# Autodesk Inventor assembly: Link_01_Assembly_V02
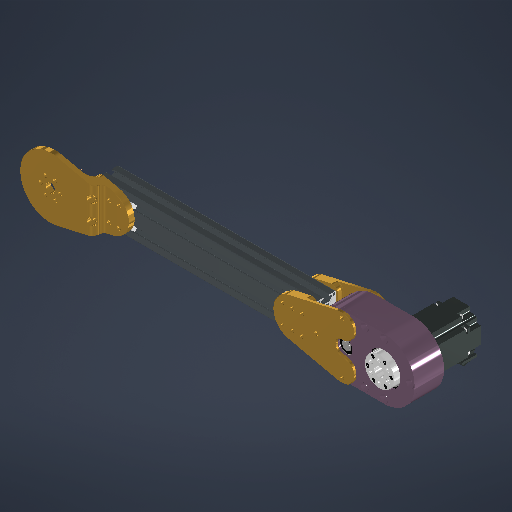
[picture p0: Inventor's stored thumbnail of the model, 512x512]
Saved by Autodesk Inventor 2026 (Build 300175000, 175)
## iProperties
Created: 2025-12-01
Part Number: Link_01_Assembly_V02
Document SubType Name: Assembly
Designer: DanielFGarzon
Mass: 2273.35 g
Surface Area: 4707.46 cm^2
Volume: 1022.63 cm^3
Density: 2.22304 g/cm^3
Author: DanielFGarzon
## Documents named in this file (5)
- D:\POLIMI\3RD SEMESTER\Industrial Robotics\Project\Mine\Link_01_Assembly_V02.iam
- D:\POLIMI\3RD SEMESTER\Industrial Robotics\Project\Mine\RotationalConector_30x60.ipt
- D:\POLIMI\3RD SEMESTER\Industrial Robotics\Project\Mine\Link_01_V02.ipt
- D:\POLIMI\3RD SEMESTER\Industrial Robotics\Project\Mine\RigidConector_30x60.ipt
- D:\POLIMI\3RD SEMESTER\Industrial Robotics\Project\Mine\Reducer.iam
## Components (5 placed, 4 different names)
1. RotationalConector_30x60:1 — Mate:1, Mate:2, Mate:3, Mate:4
2. Link_01_V02:1 — Mate:2, Mate:3, Mate:4, Mate:5, Mate:6, Mate:7, Mate:8, Mate:9, Mate:10, Flush:2, Mate:15
3. RigidConector_30x60:1 — Mate:5, Mate:6, Mate:7, Mate:11, Mate:13
4. RigidConector_30x60:2 — Mate:8, Mate:9, Mate:10, Mate:12
5. Reducer:1 [sub-assembly] — Mate:11, Mate:12, Mate:13
## Relationships (16: Mate 15, Flush 1)
- Mate:1: RotationalConector_30x60:1
- Mate:2: RotationalConector_30x60:1 ↔ Link_01_V02:1
- Mate:3: RotationalConector_30x60:1 ↔ Link_01_V02:1
- Mate:4: RotationalConector_30x60:1 ↔ Link_01_V02:1
- Mate:5: Link_01_V02:1 ↔ RigidConector_30x60:1
- Mate:6: Link_01_V02:1 ↔ RigidConector_30x60:1
- Mate:7: Link_01_V02:1 ↔ RigidConector_30x60:1
- Mate:8: Link_01_V02:1 ↔ RigidConector_30x60:2
- Mate:9: Link_01_V02:1 ↔ RigidConector_30x60:2
- Mate:10: Link_01_V02:1 ↔ RigidConector_30x60:2
- Mate:11: RigidConector_30x60:1 ↔ Reducer:1
- Mate:12: RigidConector_30x60:2 ↔ Reducer:1
- Mate:13: RigidConector_30x60:1 ↔ Reducer:1
- Flush:2 (-30 mm): Link_01_V02:1
- Mate:14
- Mate:15: Link_01_V02:1
